# Autodesk Inventor assembly: 3000_Sample Assembly_V2
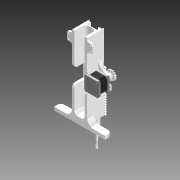
[picture p0: Inventor's stored thumbnail of the model, 180x180]
Saved by Autodesk Inventor 2021 (Build 250183000, 183)
## iProperties
Created: 2019-11-07
Part Number: 3000_Sample Assembly_V2
Document SubType Name: Assembly
Designer: RFLab
Author: RFLab
## Documents named in this file (8)
- C:\Users\RFLab\Documents\GitHub\MPS\Inventor Parts\Version 1\3xxx_Sample Assembly\3000_Sample Assembly_V2.iam
- C:\Users\RFLab\Documents\GitHub\MPS\Inventor Parts\Version 1\3xxx_Sample Assembly\32xx_ Motor and Driving\321x_Stepper Motor Parts\3211_Stepper Motor_V1.ipt
- C:\Users\RFLab\Documents\GitHub\MPS\Inventor Parts\Version 1\3xxx_Sample Assembly\31xx_Sample Rails\3101_Sample Rail Base_V1.ipt
- C:\Users\RFLab\Documents\GitHub\MPS\Inventor Parts\Version 1\3xxx_Sample Assembly\32xx_ Motor and Driving\322x_Motor Mechanical Connectors\3221_Motor Pinion_V1.ipt
- C:\Users\RFLab\Documents\GitHub\MPS\Inventor Parts\Version 1\3xxx_Sample Assembly\31xx_Sample Rails\3104_Example Bulb_V1.ipt
- C:\Users\RFLab\Documents\GitHub\MPS\Inventor Parts\Version 1\3xxx_Sample Assembly\31xx_Sample Rails\3102_Dovetail Slider_V2.ipt
- C:\Users\RFLab\Documents\GitHub\MPS\Inventor Parts\Version 1\3xxx_Sample Assembly\32xx_ Motor and Driving\322x_Motor Mechanical Connectors\3221_Motor Pinion_V3.ipt
- C:\Users\RFLab\Documents\GitHub\MPS\Inventor Parts\Version 1\3xxx_Sample Assembly\31xx_Sample Rails\3103_Bulb Arm_V4.ipt
## Components (7 placed, 7 different names)
1. 3101_Sample Rail Base_V1:1 — Mate:1, Mate:2, Mate:13, Mate:14, Mate:15, Flush:3, Mate:17, Flush:4
2. 3102_Dovetail Slider_V2:1 — Mate:1, Mate:2, Mate:23, Flush:5, Mate:24
3. 3211_Stepper Motor_V1:1 — Flush:3, Mate:17, Mate:21, Mate:22, Rotational:1, Flush:4
4. 3221_Motor Pinion_V1:1 — Mate:21, Mate:22
5. 3104_Example Bulb_V1:1 — Mate:25, Mate:26
6. Spur Gear1:1 — Rotational:1
7. 3103_Bulb Arm_V4:1 — Mate:23, Flush:5, Mate:24, Mate:25, Mate:26
## Relationships (16: Mate 12, Flush 3, RevoluteJoint 1)
- Mate:1: 3101_Sample Rail Base_V1:1 ↔ 3102_Dovetail Slider_V2:1
- Mate:2 (-0.3 mm): 3101_Sample Rail Base_V1:1 ↔ 3102_Dovetail Slider_V2:1
- Mate:13: 3101_Sample Rail Base_V1:1
- Mate:14: 3101_Sample Rail Base_V1:1
- Mate:15: 3101_Sample Rail Base_V1:1
- Flush:3: 3101_Sample Rail Base_V1:1 ↔ 3211_Stepper Motor_V1:1
- Mate:17: 3101_Sample Rail Base_V1:1 ↔ 3211_Stepper Motor_V1:1
- Mate:21: 3211_Stepper Motor_V1:1 ↔ 3221_Motor Pinion_V1:1
- Mate:22: 3211_Stepper Motor_V1:1 ↔ 3221_Motor Pinion_V1:1
- Rotational:1 [RevoluteJoint] (5 mm): 3211_Stepper Motor_V1:1 ↔ Spur Gear1:1
- Flush:4: 3101_Sample Rail Base_V1:1 ↔ 3211_Stepper Motor_V1:1
- Mate:23: 3102_Dovetail Slider_V2:1 ↔ 3103_Bulb Arm_V4:1
- Flush:5: 3102_Dovetail Slider_V2:1 ↔ 3103_Bulb Arm_V4:1
- Mate:24: 3102_Dovetail Slider_V2:1 ↔ 3103_Bulb Arm_V4:1
- Mate:25: 3104_Example Bulb_V1:1 ↔ 3103_Bulb Arm_V4:1
- Mate:26 (-2 mm): 3104_Example Bulb_V1:1 ↔ 3103_Bulb Arm_V4:1
